# Autodesk Inventor assembly: Scrambler II
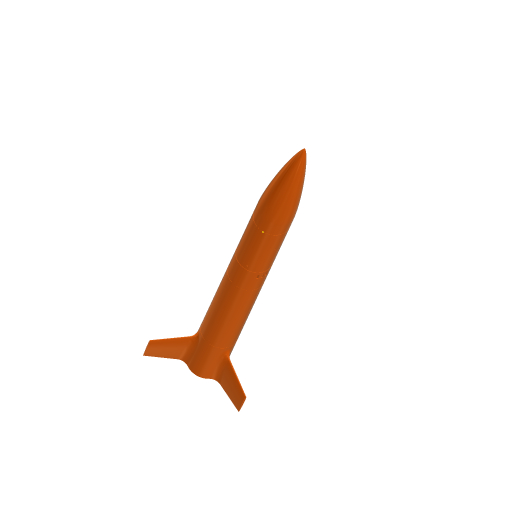
[picture p0: Inventor's stored thumbnail of the model, 512x512]
Saved by Autodesk Inventor 2024 (Build 280153000, 153)
## iProperties
Created: 2023-12-30
Part Number: Scrambler II
Document SubType Name: Assembly
Designer: Jamie
Mass: 631.455 g
Surface Area: 5625.65 cm^2
Volume: 391.502 cm^3
Density: 1.6129 g/cm^3
Author: Jamie
## Documents named in this file (5)
- C:\Users\Jamie\Documents\Uni\DARE\Scrambler-2-CAD\Hide and seek\Dummy Scrambler.iam
- C:\Users\Jamie\Documents\Uni\DARE\Scrambler-2-CAD\Hide and seek\Upper skin.ipt
- C:\Users\Jamie\Documents\Uni\DARE\Scrambler-2-CAD\Hide and seek\Nosecone.ipt
- C:\Users\Jamie\Documents\Uni\DARE\Scrambler-2-CAD\Hide and seek\Engine skin glued.iam
- Engine skin.iam
## Components (3 placed, 3 different names)
1. Upper skin:1 — Mate:10, Mate:12, Mate:13, Mate:14, Mate:15, Mate:16
2. Nosecone:1 — Mate:14, Mate:15, Mate:16
3. Engine skin:1 [sub-assembly] — Mate:10, Mate:12, Mate:13
## Relationships (6: Mate 6)
- Mate:10: Upper skin:1 ↔ Engine skin:1
- Mate:12: Upper skin:1 ↔ Engine skin:1
- Mate:13: Upper skin:1 ↔ Engine skin:1
- Mate:14: Upper skin:1 ↔ Nosecone:1
- Mate:15: Upper skin:1 ↔ Nosecone:1
- Mate:16: Upper skin:1 ↔ Nosecone:1
